# Autodesk Inventor assembly: Assembly1
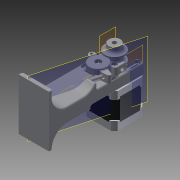
[picture p0: Inventor's stored thumbnail of the model, 180x180]
Saved by Autodesk Inventor 2015 SP1 (Build 190203100, 203)
## iProperties
Created: 2015-06-16
Part Number: Assembly1
Document SubType Name: Assembly
Designer: pc
Author: pc
## Documents named in this file (8)
- C:\Users\pc\Desktop\tractora\Assembly1.iam
- C:\Users\pc\Desktop\tractora\Imported Components\NEMA-17_Stepper_Motor_47mm\NEMA-17_Stepper_Motor_47mm.ipt
- C:\Users\pc\Desktop\tractora\pieza.rodamiento.ipt
- C:\Users\pc\Desktop\tractora\eje-largo-0.3.ipt
- C:\Users\pc\Desktop\tractora\soporte.ipt
- C:\Users\pc\Desktop\tractora\MUELLE.ipt
- C:\Users\pc\Desktop\tractora\rodamiento0.2.ipt
- C:\Users\pc\Desktop\tractora\guia.tractora.ipt
## Components (7 placed, 7 different names)
1. NEMA-17_Stepper_Motor_47mm:1 — Insert:6, Insert:9, Insert:10
2. eje-largo-0.3:1 — Insert:9
3. soporte:1 — Insert:6, Insert:7
4. MUELLE:1
5. rodamiento0.2:1 — Insert:7, Insert:8
6. pieza.rodamiento:1 — Insert:8
7. guia.tractora:1 — Insert:10
## Relationships (5: Insert 5)
- Insert:6: NEMA-17_Stepper_Motor_47mm:1 ↔ soporte:1
- Insert:7: soporte:1 ↔ rodamiento0.2:1
- Insert:8: rodamiento0.2:1 ↔ pieza.rodamiento:1
- Insert:9: NEMA-17_Stepper_Motor_47mm:1 ↔ eje-largo-0.3:1
- Insert:10 (14 mm): NEMA-17_Stepper_Motor_47mm:1 ↔ guia.tractora:1
